# Autodesk Inventor assembly: Body
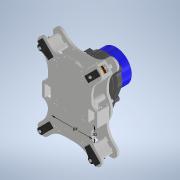
[picture p0: Inventor's stored thumbnail of the model, 180x180]
Saved by Autodesk Inventor 2020.3 (Build 243373000, 373)
## iProperties
Created: 2022-03-31
Part Number: Body
Document SubType Name: Assembly
Designer: sanyi
Author: sanyi
## Documents named in this file (8)
- C:\Users\sanyi\Documents\Inventor\Quadropod\Quadropod MDL\SimulationModell_Assembly\Body.iam
- C:\Users\sanyi\Documents\Inventor\Quadropod\BaseBottom_v1.ipt
- C:\Users\sanyi\Documents\Inventor\Quadropod\BaseTop_v1.ipt
- C:\Users\sanyi\Documents\Inventor\Quadropod\LegPin_Middle_v1.ipt
- C:\Users\sanyi\Documents\Inventor\Quadropod\LegPin_Side_v1.ipt
- C:\Users\sanyi\Documents\Inventor\Quadropod\LegPin_Side_v1_MIR.ipt
- C:\Users\sanyi\Documents\Inventor\Quadropod\SH-0257MG.ipt
- C:\Users\sanyi\Documents\Inventor\Quadropod\ydlidar x4.ipt
## Components (13 placed, 7 different names)
1. BaseBottom_v1:1 — Insert:1, Insert:2, Insert:3, Insert:4, Insert:5, Insert:6, Insert:7, Insert:8, Insert:9, Insert:10, Insert:11, Insert:12, Insert:17, Angle:1, Insert:18, Insert:19, Insert:20, Angle:2, Angle:3, Angle:4, Flush:1, Flush:2, Flush:3
2. BaseTop_v1:1 — Insert:13, Insert:14, Insert:15, Insert:16
3. LegPin_Middle_v1:1 — Insert:5, Insert:6, Insert:13
4. LegPin_Side_v1:1 — Insert:1, Insert:2
5. LegPin_Side_v1_MIR:1 — Insert:3, Insert:4
6. SH-0257MG:1 — Insert:17, Angle:1
7. ydlidar x4:1 — Insert:15, Insert:16
8. LegPin_Middle_v1:2 — Insert:7, Insert:8
9. LegPin_Middle_v1:3 — Insert:9, Insert:10, Insert:14
10. LegPin_Middle_v1:4 — Insert:11, Insert:12
11. SH-0257MG:2 — Insert:18, Angle:3
12. SH-0257MG:3 — Insert:19, Angle:4
13. SH-0257MG:4 — Insert:20, Angle:2
## Relationships (30: Insert 20, Angle 4, Flush 3, Mate 3)
- Insert:1: BaseBottom_v1:1 ↔ LegPin_Side_v1:1
- Insert:2: BaseBottom_v1:1 ↔ LegPin_Side_v1:1
- Insert:3: BaseBottom_v1:1 ↔ LegPin_Side_v1_MIR:1
- Insert:4: BaseBottom_v1:1 ↔ LegPin_Side_v1_MIR:1
- Insert:5: BaseBottom_v1:1 ↔ LegPin_Middle_v1:1
- Insert:6: BaseBottom_v1:1 ↔ LegPin_Middle_v1:1
- Insert:7: BaseBottom_v1:1 ↔ LegPin_Middle_v1:2
- Insert:8: BaseBottom_v1:1 ↔ LegPin_Middle_v1:2
- Insert:9: BaseBottom_v1:1 ↔ LegPin_Middle_v1:3
- Insert:10: BaseBottom_v1:1 ↔ LegPin_Middle_v1:3
- Insert:11: BaseBottom_v1:1 ↔ LegPin_Middle_v1:4
- Insert:12: BaseBottom_v1:1 ↔ LegPin_Middle_v1:4
- Insert:13: BaseTop_v1:1 ↔ LegPin_Middle_v1:1
- Insert:14: BaseTop_v1:1 ↔ LegPin_Middle_v1:3
- Insert:15: BaseTop_v1:1 ↔ ydlidar x4:1
- Insert:16: BaseTop_v1:1 ↔ ydlidar x4:1
- Insert:17: BaseBottom_v1:1 ↔ SH-0257MG:1
- Angle:1 (180 deg): BaseBottom_v1:1 ↔ SH-0257MG:1
- Insert:18: BaseBottom_v1:1 ↔ SH-0257MG:2
- Insert:19: BaseBottom_v1:1 ↔ SH-0257MG:3
- Insert:20: BaseBottom_v1:1 ↔ SH-0257MG:4
- Angle:2 (0 deg): BaseBottom_v1:1 ↔ SH-0257MG:4
- Angle:3 (0 deg): BaseBottom_v1:1 ↔ SH-0257MG:2
- Angle:4 (0 deg): BaseBottom_v1:1 ↔ SH-0257MG:3
- Flush:1 (-67.5 mm): BaseBottom_v1:1
- Flush:2 (-57.2 mm): BaseBottom_v1:1
- Mate:2
- Mate:3
- Flush:3 (14.58 mm): BaseBottom_v1:1
- Mate:4
